# Autodesk Inventor assembly: robo-gardener
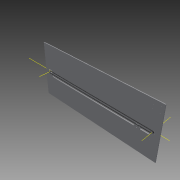
[picture p0: Inventor's stored thumbnail of the model, 180x180]
Saved by Autodesk Inventor 2013 (Build 170138000, 138)
## iProperties
Created: 2013-05-07
Part Number: robo-gardener
Document SubType Name: Assembly
Designer: Administrator
Author: Administrator
## Documents named in this file (6)
- \\vmware-host\Shared Folders\Dropbox\projects\robo-gardener\robo-gardener.iam
- \\vmware-host\Shared Folders\Dropbox\projects\robo-gardener\back-plate.ipt
- \\vmware-host\Shared Folders\Dropbox\projects\robo-gardener\robo-gardener\Design Accelerator\Synchronous Belts Transmission2.iam
- \\vmware-host\Shared Folders\Dropbox\projects\robo-gardener\carraige-face.ipt
- \\vmware-host\Shared Folders\Dropbox\projects\robo-gardener\wheel.ipt
- \\vmware-host\Shared Folders\Dropbox\projects\robo-gardener\carraige-back.ipt
## Components (6 placed, 5 different names)
1. back-plate:1 — Mate:1, Mate:2, Flush:1, Flush:2, Tangent:1, Tangent:2
2. Synchronous Belts Transmission:1 [sub-assembly]
3. carraige-face:1 — Flush:1, Flush:2, Insert:1, Insert:2
4. wheel:1 — Insert:1, Tangent:2, Insert:4
5. wheel:2 — Insert:2, Tangent:1, Insert:3
6. carraige-back:1 — Insert:3, Insert:4
## Relationships (10: Insert 4, Mate 2, Flush 2, Tangent 2)
- Mate:1: back-plate:1
- Mate:2: back-plate:1
- Flush:1: back-plate:1 ↔ carraige-face:1
- Flush:2: back-plate:1 ↔ carraige-face:1
- Insert:1: carraige-face:1 ↔ wheel:1
- Insert:2: carraige-face:1 ↔ wheel:2
- Tangent:1: back-plate:1 ↔ wheel:2
- Tangent:2: back-plate:1 ↔ wheel:1
- Insert:3: wheel:2 ↔ carraige-back:1
- Insert:4: wheel:1 ↔ carraige-back:1
